# Autodesk Inventor assembly: Inner
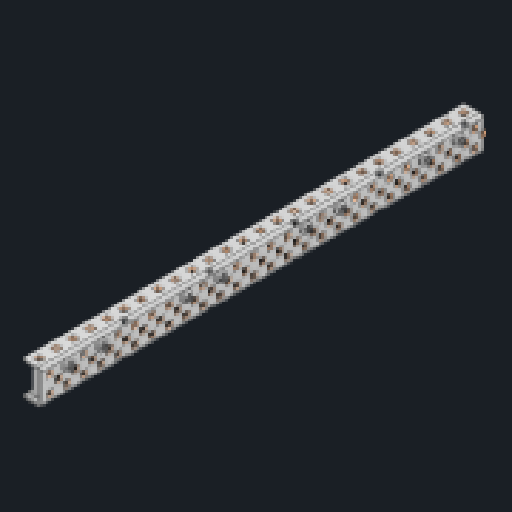
[picture p0: Inventor's stored thumbnail of the model, 512x512]
Saved by Autodesk Inventor 2025 (Build 290162000, 162)
## iProperties
Created: 2024-12-17
Part Number: Inner
Document SubType Name: Assembly
Designer: Averey Ku
Author: Averey Ku
## Documents named in this file (6)
- D:\VEX\High Stakes\CAD\V4\Chassis\Drivebay Left\Inner.iam
- D:\VEX\High Stakes\CAD\ROBOPROS-CAD-Inventor\Structure\C Channel\Aluminum 1x2x1\Alu C 1x2x1x26.ipt
- D:\VEX\High Stakes\CAD\ROBOPROS-CAD-Inventor\Structure\Nylon Standoff Rounded\Nylon Standoff .875.ipt
- D:\VEX\High Stakes\CAD\ROBOPROS-CAD-Inventor\Motion\Shaft LS\Bearing Flat Low Profile.ipt
- D:\VEX\High Stakes\CAD\ROBOPROS-CAD-Inventor\Structure\Hardware\Nut Nylon Thread-Forming.ipt
- D:\VEX\High Stakes\CAD\ROBOPROS-CAD-Inventor\Structure\Hardware\Screw Nylon - Pan Head\NScrew Pan Head Threaded .500.ipt
## Components (22 placed, 5 different names)
1. Alu C 1x2x1x26:1 — Flush:1, Flush:2, Flush:3, Insert:1, Insert:4, Mate:1, Insert:5, Insert:6
2. Nylon Standoff .875:1 — Insert:1
3. Bearing Flat Low Profile:1 — Insert:2, Insert:3, Insert:4, Mate:1
4. Nut Nylon Thread-Forming:1 — Insert:2
5. Nut Nylon Thread-Forming:2 — Insert:3
6. NScrew Pan Head Threaded .500:1 — Insert:5
7. NScrew Pan Head Threaded .500:2 — Insert:6
8. Bearing Flat Low Profile:2
9. Nut Nylon Thread-Forming:3
10. Nut Nylon Thread-Forming:4
11. NScrew Pan Head Threaded .500:3
12. NScrew Pan Head Threaded .500:4
13. Bearing Flat Low Profile:3
14. Nut Nylon Thread-Forming:5
15. Nut Nylon Thread-Forming:6
16. NScrew Pan Head Threaded .500:5
17. NScrew Pan Head Threaded .500:6
18. Bearing Flat Low Profile:4
19. Nut Nylon Thread-Forming:7
20. Nut Nylon Thread-Forming:8
21. NScrew Pan Head Threaded .500:7
22. NScrew Pan Head Threaded .500:8
## Component patterns: (4 elements, first: Bearing Flat Low Profile:1 + Nut Nylon Thread-Forming:1 + Nut Nylon Thread-Forming:2 + NScrew Pan Head Threaded .500:1 + NScrew Pan Head Threaded .500:2)
## Relationships (10: Insert 6, Flush 3, Mate 1)
- Flush:1 (-165.1 mm): Alu C 1x2x1x26:1
- Flush:2 (-7.9375 mm): Alu C 1x2x1x26:1
- Flush:3 (-12.7 mm): Alu C 1x2x1x26:1
- Insert:1: Alu C 1x2x1x26:1 ↔ Nylon Standoff .875:1
- Insert:2 (1.27 mm): Bearing Flat Low Profile:1 ↔ Nut Nylon Thread-Forming:1
- Insert:3 (1.27 mm): Bearing Flat Low Profile:1 ↔ Nut Nylon Thread-Forming:2
- Insert:4: Alu C 1x2x1x26:1 ↔ Bearing Flat Low Profile:1
- Mate:1: Alu C 1x2x1x26:1 ↔ Bearing Flat Low Profile:1
- Insert:5: Alu C 1x2x1x26:1 ↔ NScrew Pan Head Threaded .500:1
- Insert:6: Alu C 1x2x1x26:1 ↔ NScrew Pan Head Threaded .500:2
